# Autodesk Inventor assembly: Square_cell
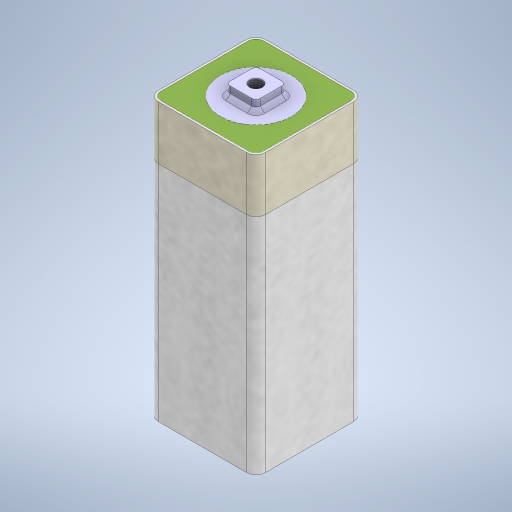
[picture p0: Inventor's stored thumbnail of the model, 512x512]
Saved by Autodesk Inventor 2023 (Build 270158000, 158)
## iProperties
Created: 2022-09-20
Part Number: Square_cell
Document SubType Name: Assembly
Designer: Makar
Mass: 934.998 g
Surface Area: 1987.7 cm^2
Volume: 289.027 cm^3
Density: 3.23499 g/cm^3
Author: Makar
## Documents named in this file (17)
- D:\NEXT SPACE Lab\NaS battery\FINAL PROJECT\Square_cell.iam
- D:\NEXT SPACE Lab\NaS battery\Metal_insert.ipt
- D:\NEXT SPACE Lab\NaS battery\Sodium_electrode.ipt
- D:\NEXT SPACE Lab\NaS battery\Solid_electrolyte.ipt
- D:\NEXT SPACE Lab\NaS battery\Cap.ipt
- D:\NEXT SPACE Lab\NaS battery\Труба 50x50x3 -110 ГОСТ 8639-82.ipt
- D:\NEXT SPACE Lab\NaS battery\Cap_top.ipt
- D:\NEXT SPACE Lab\NaS battery\Top_contact.ipt
- D:\NEXT SPACE Lab\NaS battery\Bottom_contact.ipt
- D:\NEXT SPACE Lab\NaS battery\Sulfur_electrode.ipt
- D:\NEXT SPACE Lab\NaS battery\Fiberglass_isolation.ipt
- D:\NEXT SPACE Lab\NaS battery\Square_cell\AIP\FEA\e3r9jv0m8.fins
- D:\NEXT SPACE Lab\NaS battery\Square_cell\AIP\FEA\e3r9jv0m8.fsat
- D:\NEXT SPACE Lab\NaS battery\Square_cell\AIP\FEA\e3r9jv0m8.ftes
- D:\NEXT SPACE Lab\NaS battery\Square_cell\AIP\FEA\e3r9jv0m8.fwiz
- D:\NEXT SPACE Lab\NaS battery\Square_cell\AIP\FEA\e3r9jv0u8.fmsh
- D:\NEXT SPACE Lab\NaS battery\Square_cell\AIP\FEA\e3r9jv0v4.fres
## Components (10 placed, 10 different names)
1. Metal_insert:1 — Жесткий:1, Жесткий:2
2. Sodium_electrode:1 — Жесткий:1, Жесткий:3, Жесткий:6
3. Solid_electrolyte:1 — Жесткий:2
4. Cap:1 — Жесткий:3, Жесткий:4, С поворотом:1
5. Труба 50x50x3 -110 ГОСТ 8639-82:1 — Жесткий:4, Жесткий:5, Жесткий:7
6. Cap_top:1 — Жесткий:5
7. Top_contact:1 — Жесткий:6
8. Bottom_contact:1 — Жесткий:7, Жесткий:8
9. Sulfur_electrode:1 — С поворотом:1
10. Fiberglass_isolation:1 — Жесткий:8
## Relationships (9: WeldJoint 8, RevoluteJoint 1)
- Жесткий:1 [WeldJoint] (-3 mm): Metal_insert:1 ↔ Sodium_electrode:1
- Жесткий:2 [WeldJoint]: Metal_insert:1 ↔ Solid_electrolyte:1
- Жесткий:3 [WeldJoint]: Sodium_electrode:1 ↔ Cap:1
- Жесткий:4 [WeldJoint]: Cap:1 ↔ Труба 50x50x3 -110 ГОСТ 8639-82:1
- Жесткий:5 [WeldJoint]: Труба 50x50x3 -110 ГОСТ 8639-82:1 ↔ Cap_top:1
- Жесткий:6 [WeldJoint]: Sodium_electrode:1 ↔ Top_contact:1
- Жесткий:7 [WeldJoint]: Труба 50x50x3 -110 ГОСТ 8639-82:1 ↔ Bottom_contact:1
- С поворотом:1 [RevoluteJoint]: Cap:1 ↔ Sulfur_electrode:1
- Жесткий:8 [WeldJoint]: Bottom_contact:1 ↔ Fiberglass_isolation:1
## Named parameters: sa_0 = 150000
note: some values were not read from the file. Shown as the stored number, unit unknown: "sa_0".
